# Autodesk Inventor assembly: Enclosure Assembly
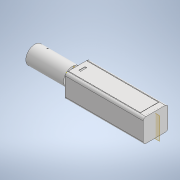
[picture p0: Inventor's stored thumbnail of the model, 180x180]
Saved by Autodesk Inventor 2022 (Build 260153000, 153)
## iProperties
Created: 2021-10-08
Part Number: Enclosure Assembly
Document SubType Name: Assembly
Designer: tecware
Author: tecware
## Documents named in this file (7)
- C:\Users\tecware\Documents\Inventor\activeMarker\wand\Base Enclosure\Enclosure Assembly.iam
- C:\Users\tecware\Documents\Inventor\activeMarker\LM2596 Buck Converter.ipt
- C:\Users\tecware\Documents\Inventor\activeMarker\Lipo.ipt
- C:\Users\tecware\Documents\Inventor\activeMarker\SPDT Switch.ipt
- C:\Users\tecware\Documents\Inventor\activeMarker\wand\Base Enclosure\battery and buck converter enclosure.ipt
- C:\Users\tecware\Documents\Inventor\activeMarker\wand\Threaded Base Attachment\thread-f.ipt
- C:\Users\tecware\Documents\Inventor\activeMarker\wand\Base Enclosure\enclosure cover.ipt
## Components (6 placed, 6 different names)
1. LM2596 Buck Converter:1
2. Lipo:1
3. SPDT Switch:1
4. battery and buck converter enclosure:1 — Flush:2, Flush:3, Flush:4, Mate:1
5. thread-f:1 — Mate:1
6. enclosure cover:1 — Flush:2, Flush:3, Flush:4
## Relationships (4: Flush 3, Mate 1)
- Flush:2 (-19.5 mm): battery and buck converter enclosure:1 ↔ enclosure cover:1
- Flush:3: battery and buck converter enclosure:1 ↔ enclosure cover:1
- Flush:4: battery and buck converter enclosure:1 ↔ enclosure cover:1
- Mate:1: battery and buck converter enclosure:1 ↔ thread-f:1
